# Autodesk Inventor assembly: 1121_Shift Coils SubAssembly_V1
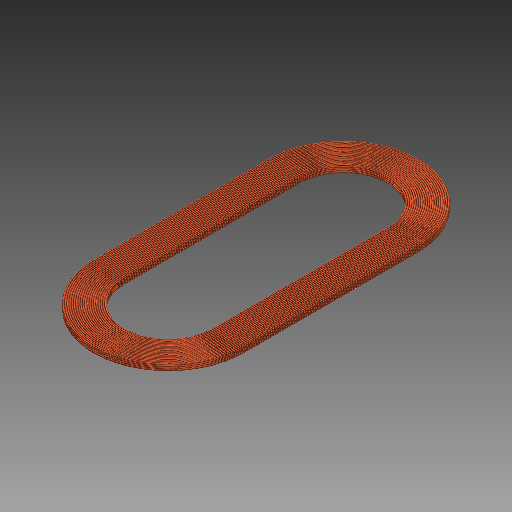
[picture p0: Inventor's stored thumbnail of the model, 512x512]
Saved by Autodesk Inventor 2020 (Build 240168000, 168)
## iProperties
Created: 2019-10-13
Part Number: 1121_Shift Coils SubAssembly_V1
Document SubType Name: Assembly
Designer: RFLab
Author: RFLab
## Documents named in this file (2)
- C:\Users\RFLab\Dropbox\MPI Group Folder\fMPI (Rodent)\Small Bore Imager_Open Source Files\Inventor Files\1xxx_Rotating Gantry\11xx_Magnet Assembly\112x_Shift Coil Assembly\1121_Shift Coils SubAssembly_V1.iam
- C:\Users\RFLab\Dropbox\MPI Group Folder\fMPI (Rodent)\Small Bore Imager_Open Source Files\Inventor Files\1xxx_Rotating Gantry\11xx_Magnet Assembly\112x_Shift Coil Assembly\1121A_Shift Coil Layer_V1.ipt
## Components (4 placed, 1 different names)
1. 1121A_Shift Coil Layer_V1:1 — Flush:1, Mate:1, Mate:2, Mate:3
2. 1121A_Shift Coil Layer_V1:2 — Flush:1, Flush:2, Mate:1, Flush:3, Mate:3, Flush:5
3. 1121A_Shift Coil Layer_V1:3 — Flush:2, Mate:2, Flush:3, Flush:4, Flush:5, Flush:6, Flush:7
4. 1121A_Shift Coil Layer_V1:4 — Flush:4, Flush:6, Flush:7
## Relationships (10: Flush 7, Mate 3)
- Flush:1: 1121A_Shift Coil Layer_V1:1 ↔ 1121A_Shift Coil Layer_V1:2
- Flush:2: 1121A_Shift Coil Layer_V1:2 ↔ 1121A_Shift Coil Layer_V1:3
- Mate:1: 1121A_Shift Coil Layer_V1:1 ↔ 1121A_Shift Coil Layer_V1:2
- Mate:2: 1121A_Shift Coil Layer_V1:1 ↔ 1121A_Shift Coil Layer_V1:3
- Flush:3: 1121A_Shift Coil Layer_V1:2 ↔ 1121A_Shift Coil Layer_V1:3
- Mate:3: 1121A_Shift Coil Layer_V1:1 ↔ 1121A_Shift Coil Layer_V1:2
- Flush:4: 1121A_Shift Coil Layer_V1:3 ↔ 1121A_Shift Coil Layer_V1:4
- Flush:5: 1121A_Shift Coil Layer_V1:2 ↔ 1121A_Shift Coil Layer_V1:3
- Flush:6: 1121A_Shift Coil Layer_V1:3 ↔ 1121A_Shift Coil Layer_V1:4
- Flush:7: 1121A_Shift Coil Layer_V1:3 ↔ 1121A_Shift Coil Layer_V1:4
